# Autodesk Inventor assembly: gimbal_v1
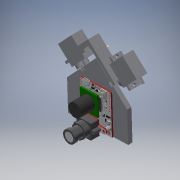
[picture p0: Inventor's stored thumbnail of the model, 180x180]
Saved by Autodesk Inventor 2019 (Build 230136000, 136)
## iProperties
Created: 2020-03-15
Part Number: gimbal_v1
Document SubType Name: Assembly
Designer: Pulag
Author: Pulag
## Documents named in this file (8)
- C:\Users\Pulag\Documents\GitHub\24th_TDK_Project_D5\CAD\frame\gimbal_v1.iam
- C:\Users\Pulag\Documents\GitHub\24th_TDK_Project_D5\CAD\Syno_borad_3D\匯出\SG90.ipt
- C:\Users\Pulag\Documents\GitHub\24th_TDK_Project_D5\CAD\frame\frame1.ipt
- C:\Users\Pulag\Documents\GitHub\24th_TDK_Project_D5\CAD\frame\frame2.ipt
- C:\Users\Pulag\Documents\GitHub\24th_TDK_Project_D5\CAD\frame\frame3.ipt
- C:\Users\Pulag\Documents\GitHub\24th_TDK_Project_D5\CAD\frame\frame4.ipt
- C:\Users\Pulag\Documents\GitHub\24th_TDK_Project_D5\CAD\CAD file\OpenMV H7\openmv4_h7.iam
- C:\Users\Pulag\Documents\GitHub\24th_TDK_Project_D5\CAD\frame\SONIC.ipt
## Components (8 placed, 7 different names)
1. SG90:1 — Rotational:1, Flush:1, Flush:2, Mate:7
2. SG90:2 — Rotational:2, Mate:10, Angle:1
3. frame1:1 — Rotational:1, Mate:8, Flush:3, Flush:4, Mate:9, Flush:5, Flush:6
4. frame2:1 — Flush:1, Flush:2, Mate:7, Rotational:2
5. frame3:1
6. frame4:1
7. openmv4_h7:1 [sub-assembly] — Mate:8, Flush:3, Flush:4
8. SONIC:1 — Mate:9, Flush:5, Flush:6
## Relationships (13: Flush 6, Mate 4, RevoluteJoint 2, Angle 1)
- Rotational:1 [RevoluteJoint]: SG90:1 ↔ frame1:1
- Flush:1: SG90:1 ↔ frame2:1
- Flush:2: SG90:1 ↔ frame2:1
- Mate:7: SG90:1 ↔ frame2:1
- Rotational:2 [RevoluteJoint]: SG90:2 ↔ frame2:1
- Mate:8: frame1:1 ↔ openmv4_h7:1
- Flush:3: frame1:1 ↔ openmv4_h7:1
- Flush:4 (-17.22 mm): frame1:1 ↔ openmv4_h7:1
- Mate:9 (8 mm): frame1:1 ↔ SONIC:1
- Flush:5 (20 mm): frame1:1 ↔ SONIC:1
- Flush:6 (25 mm): frame1:1 ↔ SONIC:1
- Mate:10: SG90:2
- Angle:1 (43 deg): SG90:2
